# Autodesk Inventor assembly: BOT Design
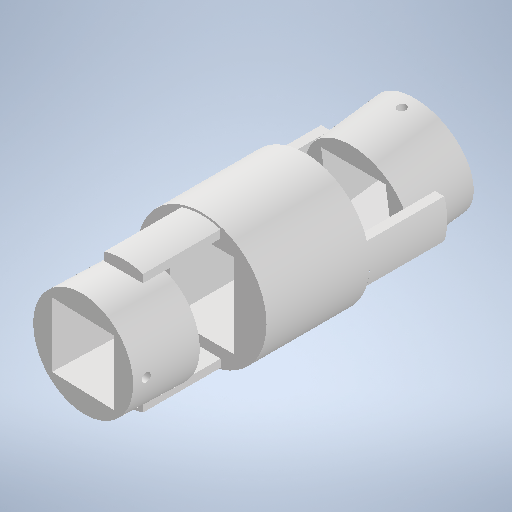
[picture p0: Inventor's stored thumbnail of the model, 512x512]
Saved by Autodesk Inventor 2025 (Build 290162000, 162)
## iProperties
Created: 2025-03-27
Part Number: BOT Design
Document SubType Name: Assembly
Designer: parsh
Author: parsh
## Documents named in this file (5)
- C:\Users\parsh\OneDrive\Documents\Disqaster Relife Bot\BOT Design.iam
- C:\Users\parsh\OneDrive\Documents\Inventor\Content Center Files\R2025\B1.ipt
- C:\Users\parsh\OneDrive\Documents\Inventor\Content Center Files\R2025\Hindge sine.ipt
- C:\Users\parsh\OneDrive\Documents\Inventor\Content Center Files\R2025\B2.ipt
- C:\Users\parsh\OneDrive\Documents\Inventor\Content Center Files\R2025\Hindge Lift.ipt
## Components (7 placed, 4 different names)
1. B1:1 — Mate:1, Mate:2, Mate:4, Mate:5
2. Hindge sine:1 — Mate:1, Mate:3
3. Hindge sine:2 — Mate:2
4. B2:1 — Mate:3
5. Hindge Lift:1 — Mate:5
6. Hindge Lift:2 — Mate:4, Mate:6
7. B2:2 — Mate:6
## Relationships (6: Mate 6)
- Mate:1: B1:1 ↔ Hindge sine:1
- Mate:2: B1:1 ↔ Hindge sine:2
- Mate:3: Hindge sine:1 ↔ B2:1
- Mate:4: B1:1 ↔ Hindge Lift:2
- Mate:5: B1:1 ↔ Hindge Lift:1
- Mate:6: Hindge Lift:2 ↔ B2:2
